# Autodesk Inventor assembly: Hafele Rafix Connector
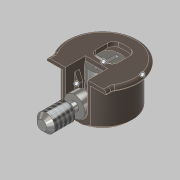
[picture p0: Inventor's stored thumbnail of the model, 180x180]
Saved by Autodesk Inventor 2022.3 (Build 263350030, 350C)
## iProperties
Created: 2023-03-10
Part Number: Hafele Rafix Connector
Document SubType Name: Assembly
Designer: S. Dereskevicius
Description: Hafele Rafix Connector
Author: sauliusd
## iProperties of the stored document MemberDocs/x2onwzwytKc1t5scn4zcrb24y4d
Created: 2023-03-10
Part Number: Hafele Rafix Connector
Document SubType Name: Assembly
Designer: S. Dereskevicius
Description: Hafele Rafix Connector
Author: sauliusd
## iProperties of the stored document MemberDocs/x22iiy1idJc4l0lncAxjzeun2Wd
Created: 2023-03-10
Part Number: Hafele Rafix Connector
Description: Hafele Rafix Connector
Document SubType Name: Assembly
Designer: S. Dereskevicius
Author: sauliusd
## iProperties of the stored document MemberDocs/xBza4go3pMcmfemkvMzi31zrnPh
Created: 2023-03-10
Part Number: Hafele Rafix Connector
Document SubType Name: Assembly
Designer: S. Dereskevicius
Description: Hafele Rafix Connector
Author: sauliusd
## iProperties of the stored document MemberDocs/x3pm4xy0uG04ffb1tEnglz5mlYa
Created: 2023-03-10
Part Number: Hafele Rafix Connector
Description: Hafele Rafix Connector
Document SubType Name: Assembly
Designer: S. Dereskevicius
Author: sauliusd
## iProperties of the stored document MemberDocs/xQatxa4bbEchp31tjOuol3heeGa
Created: 2023-03-10
Part Number: Hafele Rafix Connector
Description: Hafele Rafix Connector
Document SubType Name: Assembly
Designer: S. Dereskevicius
Author: sauliusd
## iProperties of the stored document MemberDocs/xGifgu5jkBccmcbosJkolef23Vg
Created: 2023-03-10
Part Number: Hafele Rafix Connector
Document SubType Name: Assembly
Designer: S. Dereskevicius
Description: Hafele Rafix Connector
Author: sauliusd
## iProperties of the stored document MemberDocs/xXtyp1mgyAswbk54uMupzuvuuXh
Created: 2023-03-10
Part Number: Hafele Rafix Connector
Description: Hafele Rafix Connector
Document SubType Name: Assembly
Designer: S. Dereskevicius
Author: sauliusd
## Documents named in this file (7)
- C:\W4INV 2024 Design\PROJECTS\MODEL STATE LIBRARY COMPONENTS\Rafix S20\Rafix.iam
- C:\W4INV 2022 Design\PROJECTS\Rafix\Rafix.ipt
- C:\W4INV 2022 Design\PROJECTS\Rafix\Rafix Bolt.ipt
- C:\W4INV 2024 Design\PROJECTS\MODEL STATE LIBRARY COMPONENTS\Rafix S20\Parts\Rafix.ipt
- C:\W4INV 2024 Design\PROJECTS\MODEL STATE LIBRARY COMPONENTS\Rafix S20\Parts\Rafix Bolt.ipt
- C:\W4INV 2023 Design\PROJECTS\MODEL STATE LIBRARY COMPONENTS\Rafix S20\Parts\Rafix.ipt
- C:\W4INV 2023 Design\PROJECTS\MODEL STATE LIBRARY COMPONENTS\Rafix S20\Parts\Rafix Bolt.ipt
## Components (2 placed, 2 different names)
1. Rafix:1 — Mate:1, Mate:3
2. Rafix Bolt:1 — Mate:1, Mate:2, Mate:3
## Relationships (3: Mate 3)
- Mate:1: Rafix:1 ↔ Rafix Bolt:1
- Mate:2: Rafix Bolt:1
- Mate:3: Rafix:1 ↔ Rafix Bolt:1
## Named parameters: NestledBoardT = 18 mm, PillarBoardT = 18 mm
